# Autodesk Inventor assembly: Standformiddleslide
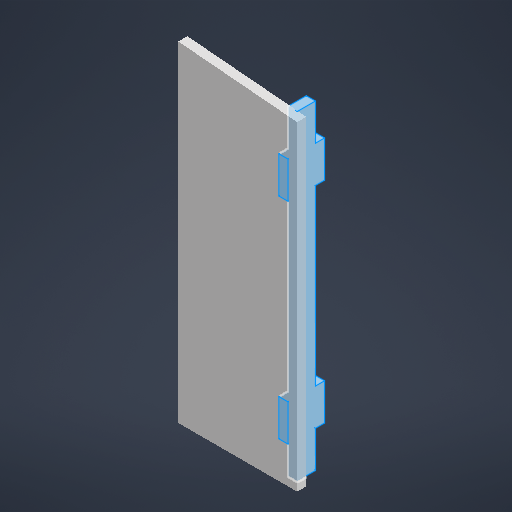
[picture p0: Inventor's stored thumbnail of the model, 512x512]
Saved by Autodesk Inventor 2026.2 (Build 302298000, 298)
## iProperties
Created: 2026-04-17
Part Number: Standformiddleslide
Document SubType Name: Assembly
Designer: danda
Author: danda
## Documents named in this file (3)
- C:\Users\danda\BOM-project\Project\CAD\sorting\Standformiddleslide.iam
- C:\Users\danda\BOM-project\Project\CAD\sorting\stand.ipt
- C:\Users\danda\BOM-project\Project\CAD\sorting\standformiddleslide2.ipt
## Components (2 placed, 2 different names)
1. stand:1 — Mate:1, Mate:2, Flush:1
2. standformiddleslide2:1 — Mate:1, Mate:2, Flush:1
## Relationships (3: Mate 2, Flush 1)
- Mate:1: stand:1 ↔ standformiddleslide2:1
- Mate:2: stand:1 ↔ standformiddleslide2:1
- Flush:1: stand:1 ↔ standformiddleslide2:1
